# Autodesk Inventor assembly: Long AM14U3 with Bumpers and Battery Tray 2018
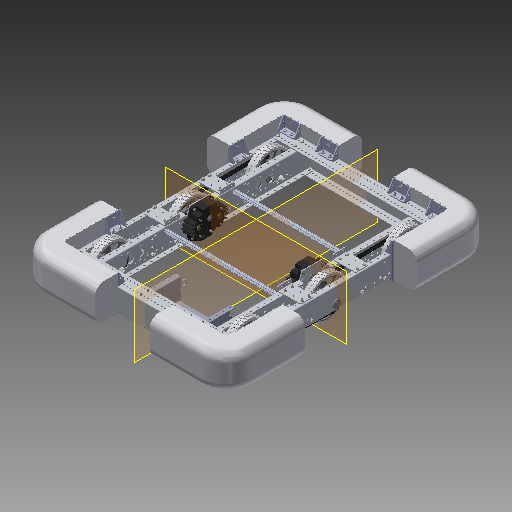
[picture p0: Inventor's stored thumbnail of the model, 512x512]
Saved by Autodesk Inventor 2019 (Build 230136000, 136)
## iProperties
Created: 2017-12-15
Part Number: Long AM14U3 with Bumpers and Battery Tray 2018
Document SubType Name: Assembly
Designer: PhillipD
Author: PhillipD
Revision Number: ANY
## Documents named in this file (9)
- C:\git\CAD-Development\robSteele\2018-FRC\AMbaseLongWithBumper\Long with Bumper\DB_DriveBaseLong_AM14U3_Bumpers and Battery Tray.iam
- C:\git\CAD-Development\robSteele\2018-FRC\AMbaseLongWithBumper\Long with Bumper\Parts\AM14U3 Long.iam
- C:\git\CAD-Development\robSteele\2018-FRC\AMbaseLongWithBumper\Long with Bumper\Parts\am-3675 - BR18 Front.Corner Bumper Bracket.ipt
- C:\git\CAD-Development\robSteele\2018-FRC\AMbaseLongWithBumper\Long with Bumper\Parts\am-3674 - BR18 Side Bumper Bracket.ipt
- C:\git\CAD-Development\robSteele\2018-FRC\AMbaseLongWithBumper\Long with Bumper\Parts\10-32x0625_shcs_HX-SHCS 0.19-32x1.375x1-C.ipt
- C:\git\CAD-Development\robSteele\2018-FRC\AMbaseLongWithBumper\Long with Bumper\Parts\10-32 Nylock Nut.ipt
- C:\git\CAD-Development\robSteele\2018-FRC\AMbaseLongWithBumper\Long with Bumper\Parts\10-32 x 1000 Thumb Screw with Washer_91744A833.ipt
- C:\git\CAD-Development\robSteele\2018-FRC\AMbaseLongWithBumper\Long with Bumper\Parts\Corner Bumper Kit.iam
- C:\git\CAD-Development\robSteele\2018-FRC\AMbaseLongWithBumper\Long with Bumper\Parts\BatteryHolder.iam
## Components (82 placed, 82 different names)
1. AM14U3 Long_129 [sub-assembly] — Flush:1, Flush:2
2. am-3675 - BR18 Front.Corner Bumper Bracket_130
3. am-3675 - BR18 Front.Corner Bumper Bracket_131
4. am-3675 - BR18 Front.Corner Bumper Bracket_132
5. am-3675 - BR18 Front.Corner Bumper Bracket_133
6. am-3675 - BR18 Front.Corner Bumper Bracket_134
7. am-3675 - BR18 Front.Corner Bumper Bracket_135
8. am-3674 - BR18 Side Bumper Bracket_136
9. am-3674 - BR18 Side Bumper Bracket_137
10. am-3674 - BR18 Side Bumper Bracket_138
11. am-3674 - BR18 Side Bumper Bracket_139
12. am-3675 - BR18 Front.Corner Bumper Bracket_140
13. am-3675 - BR18 Front.Corner Bumper Bracket_141
14. 10-32x0625_shcs_HX-SHCS 0.19-32x1.375x1-C_142
15. 10-32x0625_shcs_HX-SHCS 0.19-32x1.375x1-C_143
16. 10-32x0625_shcs_HX-SHCS 0.19-32x1.375x1-C_144
17. 10-32x0625_shcs_HX-SHCS 0.19-32x1.375x1-C_145
18. 10-32x0625_shcs_HX-SHCS 0.19-32x1.375x1-C_146
19. 10-32x0625_shcs_HX-SHCS 0.19-32x1.375x1-C_147
20. 10-32x0625_shcs_HX-SHCS 0.19-32x1.375x1-C_148
21. 10-32x0625_shcs_HX-SHCS 0.19-32x1.375x1-C_149
22. 10-32x0625_shcs_HX-SHCS 0.19-32x1.375x1-C_150
23. 10-32x0625_shcs_HX-SHCS 0.19-32x1.375x1-C_151
24. 10-32x0625_shcs_HX-SHCS 0.19-32x1.375x1-C_152
25. 10-32x0625_shcs_HX-SHCS 0.19-32x1.375x1-C_153
26. 10-32x0625_shcs_HX-SHCS 0.19-32x1.375x1-C_154
27. 10-32x0625_shcs_HX-SHCS 0.19-32x1.375x1-C_155
28. 10-32x0625_shcs_HX-SHCS 0.19-32x1.375x1-C_156
29. 10-32x0625_shcs_HX-SHCS 0.19-32x1.375x1-C_157
30. 10-32x0625_shcs_HX-SHCS 0.19-32x1.375x1-C_158
31. 10-32x0625_shcs_HX-SHCS 0.19-32x1.375x1-C_159
32. 10-32x0625_shcs_HX-SHCS 0.19-32x1.375x1-C_160
33. 10-32x0625_shcs_HX-SHCS 0.19-32x1.375x1-C_161
34. 10-32x0625_shcs_HX-SHCS 0.19-32x1.375x1-C_162
35. 10-32x0625_shcs_HX-SHCS 0.19-32x1.375x1-C_163
36. 10-32x0625_shcs_HX-SHCS 0.19-32x1.375x1-C_164
37. 10-32x0625_shcs_HX-SHCS 0.19-32x1.375x1-C_165
38. 10-32 Nylock Nut_166
39. 10-32 Nylock Nut_167
40. 10-32 Nylock Nut_168
41. 10-32 Nylock Nut_169
42. 10-32 Nylock Nut_170
43. 10-32 Nylock Nut_171
44. 10-32 Nylock Nut_172
45. 10-32 Nylock Nut_173
46. 10-32 Nylock Nut_174
47. 10-32 Nylock Nut_175
48. 10-32 Nylock Nut_176
49. 10-32 Nylock Nut_177
50. 10-32 Nylock Nut_178
51. 10-32 Nylock Nut_179
52. 10-32 Nylock Nut_180
53. 10-32 Nylock Nut_181
54. 10-32 Nylock Nut_182
55. 10-32 Nylock Nut_183
56. 10-32 Nylock Nut_184
57. 10-32 Nylock Nut_185
58. 10-32 Nylock Nut_186
59. 10-32 Nylock Nut_187
60. 10-32 Nylock Nut_188
61. 10-32 Nylock Nut_189
62. 10-32 x 1000 Thumb Screw with Washer_91744A833_190
63. 10-32 x 1000 Thumb Screw with Washer_91744A833_191
64. 10-32 x 1000 Thumb Screw with Washer_91744A833_192
65. 10-32 x 1000 Thumb Screw with Washer_91744A833_193
66. 10-32 x 1000 Thumb Screw with Washer_91744A833_194
67. 10-32 x 1000 Thumb Screw with Washer_91744A833_195
68. 10-32 x 1000 Thumb Screw with Washer_91744A833_196
69. 10-32 x 1000 Thumb Screw with Washer_91744A833_197
70. 10-32 x 1000 Thumb Screw with Washer_91744A833_198
71. 10-32 x 1000 Thumb Screw with Washer_91744A833_199
72. 10-32 x 1000 Thumb Screw with Washer_91744A833_200
73. 10-32 x 1000 Thumb Screw with Washer_91744A833_201
74. 10-32 x 1000 Thumb Screw with Washer_91744A833_202
75. 10-32 x 1000 Thumb Screw with Washer_91744A833_203
76. 10-32 x 1000 Thumb Screw with Washer_91744A833_204
77. 10-32 x 1000 Thumb Screw with Washer_91744A833_205
78. Corner Bumper Kit_206 [sub-assembly]
79. Corner Bumper Kit_207 [sub-assembly]
80. Corner Bumper Kit_208 [sub-assembly]
81. Corner Bumper Kit_209 [sub-assembly]
82. BatteryHolder_210 [sub-assembly]
## Relationships (2: Flush 2)
- Flush:1 (206.375 mm): AM14U3 Long_129
- Flush:2 (-411.607 mm): AM14U3 Long_129
